# Autodesk Inventor assembly: New_End_Effector_Assembly
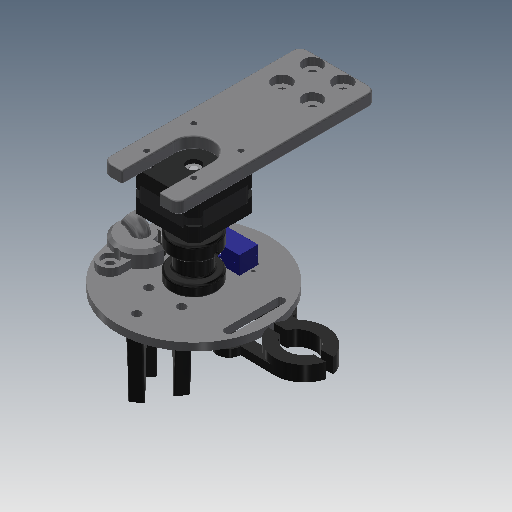
[picture p0: Inventor's stored thumbnail of the model, 512x512]
Saved by Autodesk Inventor 2020.3 (Build 243373000, 373)
## iProperties
Created: 2021-08-25
Part Number: New_End_Effector_Assembly
Document SubType Name: Assembly
Designer: justi
Author: justi
## Documents named in this file (13)
- F:\UQ Engineering\2021 ~ 5th Year\Semester 2\METR4911-THESIS\FarmBot CAD\FarmBotV1\New_End_Effector_Assembly.iam
- F:\UQ Engineering\2021 ~ 5th Year\Semester 2\METR4911-THESIS\FarmBot CAD\FarmBotV1\Rework+Simple+25_1+Cycloidal+Actuator\files\sim_nema_17\Workspaces\Workspace\NEMA17_Pancake_Motor.ipt
- F:\UQ Engineering\2021 ~ 5th Year\Semester 2\METR4911-THESIS\FarmBot CAD\FarmBotV1\New_End_Effector_Mount.ipt
- F:\UQ Engineering\2021 ~ 5th Year\Semester 2\METR4911-THESIS\FarmBot CAD\FarmBotV1\End_Effector_Coupler.ipt
- F:\UQ Engineering\2021 ~ 5th Year\Semester 2\METR4911-THESIS\FarmBot CAD\FarmBotV1\EndEffectorPlate.ipt
- F:\UQ Engineering\2021 ~ 5th Year\Semester 2\METR4911-THESIS\FarmBot CAD\FarmBotV1\tower-pro-sg90-micro-servo\microservoAssembly.iam
- F:\UQ Engineering\2021 ~ 5th Year\Semester 2\METR4911-THESIS\FarmBot CAD\FarmBotV1\EndEffectorAssembly\Design Accelerator\Spur Gears2.iam
- F:\UQ Engineering\2021 ~ 5th Year\Semester 2\METR4911-THESIS\FarmBot CAD\FarmBotV1\tower-pro-sg90-micro-servo\Rackv1.ipt
- F:\UQ Engineering\2021 ~ 5th Year\Semester 2\METR4911-THESIS\FarmBot CAD\FarmBotV1\tower-pro-sg90-micro-servo\WeedingTeeth.ipt
- F:\UQ Engineering\2021 ~ 5th Year\Semester 2\METR4911-THESIS\FarmBot CAD\FarmBotV1\tower-pro-sg90-micro-servo\DiffusionModule.ipt
- F:\UQ Engineering\2021 ~ 5th Year\Semester 2\METR4911-THESIS\FarmBot CAD\FarmBotV1\DiffusionModuleCover.ipt
- F:\UQ Engineering\2021 ~ 5th Year\Semester 2\METR4911-THESIS\FarmBot CAD\FarmBotV1\CameraMount.ipt
- F:\UQ Engineering\2021 ~ 5th Year\Semester 2\METR4911-THESIS\FarmBot CAD\FarmBotV1\CameraMount_MIR.ipt
## Components (14 placed, 12 different names)
1. NEMA17_Pancake_Motor:1 — Mate:1, Mate:2, Mate:4, Mate:33
2. New_End_Effector_Mount:1 — Mate:1, Mate:2, Flush:1, Mate:33
3. End_Effector_Coupler:1 — Mate:4, Mate:22, Mate:23, Mate:24
4. EndEffectorPlate:1 — Mate:22, Mate:23, Mate:24, Mate:25, Mate:26, Mate:29, Mate:30, Mate:31, Mate:32
5. microservoAssembly:1 [sub-assembly]
6. Spur Gears:1 [sub-assembly]
7. Rackv1:1 — Mate:25
8. WeedingTeeth:1
9. WeedingTeeth:2
10. WeedingTeeth:3
11. DiffusionModule:1 — Mate:27, Mate:28
12. DiffusionModuleCover:1 — Mate:26, Mate:27, Mate:28
13. CameraMount:1 — Mate:29, Mate:30
14. CameraMount_MIR:1 — Mate:31, Mate:32
## Relationships (31: Mate 28, Flush 3)
- Mate:1: NEMA17_Pancake_Motor:1 ↔ New_End_Effector_Mount:1
- Mate:2: NEMA17_Pancake_Motor:1 ↔ New_End_Effector_Mount:1
- Mate:4: NEMA17_Pancake_Motor:1 ↔ End_Effector_Coupler:1
- Flush:1: New_End_Effector_Mount:1
- [Mate]: EndEffectorPlate:1 ↔ microservoAssembly:1
- [Mate]: EndEffectorPlate:1 ↔ microservoAssembly:1
- [Mate]: EndEffectorPlate:1 ↔ microservoAssembly:1
- [Mate]: microservoAssembly:1 ↔ Spur Gears:1
- [Flush]: microservoAssembly:1 ↔ Spur Gears:1
- [Mate]: microservoAssembly:1 ↔ Spur Gears:1
- [Flush] (-8.5 mm): microservoAssembly:1 ↔ Rackv1:1
- [Mate]: EndEffectorPlate:1 ↔ WeedingTeeth:1
- [Mate]: EndEffectorPlate:1 ↔ WeedingTeeth:2
- [Mate]: EndEffectorPlate:1 ↔ WeedingTeeth:3
- [Mate]: EndEffectorPlate:1 ↔ WeedingTeeth:1
- [Mate]: EndEffectorPlate:1 ↔ WeedingTeeth:3
- [Mate]: EndEffectorPlate:1 ↔ WeedingTeeth:2
- [Mate]: EndEffectorPlate:1 ↔ DiffusionModule:1
- [Mate]: EndEffectorPlate:1 ↔ DiffusionModule:1
- Mate:22: End_Effector_Coupler:1 ↔ EndEffectorPlate:1
- Mate:23: End_Effector_Coupler:1 ↔ EndEffectorPlate:1
- Mate:24: End_Effector_Coupler:1 ↔ EndEffectorPlate:1
- Mate:25: EndEffectorPlate:1 ↔ Rackv1:1
- Mate:26: EndEffectorPlate:1 ↔ DiffusionModuleCover:1
- Mate:27: DiffusionModule:1 ↔ DiffusionModuleCover:1
- Mate:28: DiffusionModule:1 ↔ DiffusionModuleCover:1
- Mate:29: EndEffectorPlate:1 ↔ CameraMount:1
- Mate:30: EndEffectorPlate:1 ↔ CameraMount:1
- Mate:31: EndEffectorPlate:1 ↔ CameraMount_MIR:1
- Mate:32: EndEffectorPlate:1 ↔ CameraMount_MIR:1
- Mate:33: NEMA17_Pancake_Motor:1 ↔ New_End_Effector_Mount:1
## Named parameters: d11_d15 = 0 mm, d12_d16 = 0 mm, d13_d17 = 0 mm, d15_d21 = -8.5 mm, d16_d22 = 0 mm, d17_d23 = 0 mm
